# Autodesk Inventor assembly: link4
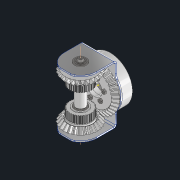
[picture p0: Inventor's stored thumbnail of the model, 180x180]
Saved by Autodesk Inventor 2021 (Build 250183000, 183)
## iProperties
Created: 2021-08-10
Part Number: link4
Document SubType Name: Assembly
Designer: yuta0
Author: yuta0
## Documents named in this file (2)
- C:\Users\yuta0\Documents\GitHub\catchrobo_hardware\mesh\link4.iam
- C:\Users\yuta0\Documents\GitHub\catchrobo_hardware\assy-robot\s-assy-link4.iam
## Components (1 placed, 1 different names)
1. s-assy-link4:1 [sub-assembly] — メイト:1, メイト:2
## Relationships (2: Mate 2)
- メイト:1 [Mate]: s-assy-link4:1
- メイト:2 [Mate]: s-assy-link4:1
